# Autodesk Inventor assembly: Sestava
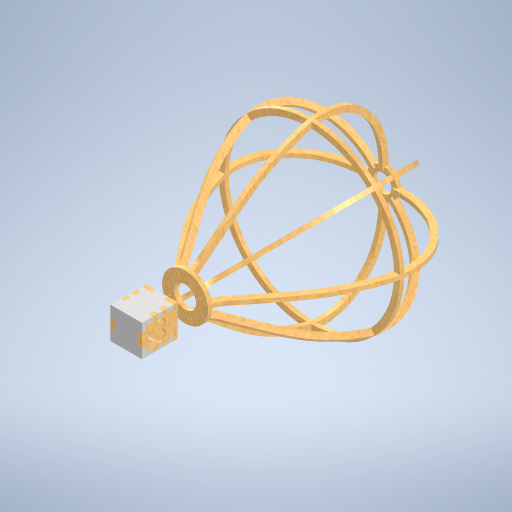
[picture p0: Inventor's stored thumbnail of the model, 512x512]
Saved by Autodesk Inventor 2023 (Build 270158000, 158)
## iProperties
Created: 2022-12-16
Part Number: Sestava
Document SubType Name: Assembly
Designer: David Zindović
Author: David Zindović
## Documents named in this file (9)
- C:\Users\David Zindović\Desktop\Projekti\Darila\Dekoracija - Balon za mami\Sestava.iam
- C:\Users\David Zindović\Desktop\Projekti\Darila\Dekoracija - Balon za mami\Sirsi obroc.ipt
- C:\Users\David Zindović\Desktop\Projekti\Darila\Dekoracija - Balon za mami\Balon skelet.ipt
- C:\Users\David Zindović\Desktop\Projekti\Darila\Dekoracija - Balon za mami\Vrhnji obrok.ipt
- C:\Users\David Zindović\Desktop\Projekti\Darila\Dekoracija - Balon za mami\Spodnji obroc.ipt
- C:\Users\David Zindović\Desktop\Projekti\Darila\Dekoracija - Balon za mami\Spodnji del - stranica.ipt
- C:\Users\David Zindović\Desktop\Projekti\Darila\Dekoracija - Balon za mami\Spodnji del - Drzalo za pismo.ipt
- C:\Users\David Zindović\Desktop\Projekti\Darila\Dekoracija - Balon za mami\Stran Stran.ipt
- C:\Users\David Zindović\Desktop\Projekti\Darila\Dekoracija - Balon za mami\Spodi Spodnji.ipt
## Components (17 placed, 8 different names)
1. Sirsi obroc:1 — Mate:1, Mate:2, Mate:3, Mate:4, Mate:5, Mate:6, Mate:7, Mate:8, Mate:9, Mate:10, Mate:11, Mate:12, Mate:13, Mate:14, Mate:15, Mate:16, Mate:17, Mate:18, Mate:19, Mate:20, Mate:21, Mate:22, Mate:23, Mate:24
2. Balon skelet:1 — Mate:8, Mate:16, Mate:20, Mate:31
3. Balon skelet:2 — Mate:7, Mate:14, Mate:22
4. Balon skelet:3 — Mate:4, Mate:10, Mate:11
5. Balon skelet:4 — Mate:3, Mate:15, Mate:21
6. Balon skelet:5 — Mate:2, Mate:17, Mate:19, Mate:30
7. Balon skelet:6 — Mate:5, Mate:18, Mate:24, Mate:32
8. Balon skelet:7 — Mate:1, Mate:9, Mate:12
9. Balon skelet:8 — Mate:6, Mate:13, Mate:23, Mate:29, Flush:1
10. Vrhnji obrok:1 — Mate:29, Mate:30
11. Spodnji obroc:1 — Mate:31, Mate:32, Flush:1
12. Spodnji del - stranica:1 — Mate:35, Mate:36, Flush:3, Flush:8, Flush:9
13. Spodnji del - stranica:2 — Mate:33, Flush:2, Mate:34
14. Spodnji del - Drzalo za pismo:1 — Mate:33, Flush:2, Mate:34, Mate:35, Mate:36, Flush:3, Mate:37, Flush:4, Flush:5, Mate:38, Flush:6, Flush:7
15. Stran Stran:1 — Mate:37, Flush:4, Flush:5
16. Stran Stran:2 — Mate:38, Flush:6, Flush:7, Flush:10
17. Spodi Spodnji:1 — Flush:8, Flush:9, Flush:10
## Relationships (44: Mate 34, Flush 10)
- Mate:1: Sirsi obroc:1 ↔ Balon skelet:7
- Mate:2: Sirsi obroc:1 ↔ Balon skelet:5
- Mate:3: Sirsi obroc:1 ↔ Balon skelet:4
- Mate:4: Sirsi obroc:1 ↔ Balon skelet:3
- Mate:5: Sirsi obroc:1 ↔ Balon skelet:6
- Mate:6: Sirsi obroc:1 ↔ Balon skelet:8
- Mate:7: Sirsi obroc:1 ↔ Balon skelet:2
- Mate:8: Sirsi obroc:1 ↔ Balon skelet:1
- Mate:9: Sirsi obroc:1 ↔ Balon skelet:7
- Mate:10: Sirsi obroc:1 ↔ Balon skelet:3
- Mate:11: Sirsi obroc:1 ↔ Balon skelet:3
- Mate:12: Sirsi obroc:1 ↔ Balon skelet:7
- Mate:13: Sirsi obroc:1 ↔ Balon skelet:8
- Mate:14: Sirsi obroc:1 ↔ Balon skelet:2
- Mate:15: Sirsi obroc:1 ↔ Balon skelet:4
- Mate:16: Sirsi obroc:1 ↔ Balon skelet:1
- Mate:17: Sirsi obroc:1 ↔ Balon skelet:5
- Mate:18: Sirsi obroc:1 ↔ Balon skelet:6
- Mate:19: Sirsi obroc:1 ↔ Balon skelet:5
- Mate:20: Sirsi obroc:1 ↔ Balon skelet:1
- Mate:21: Sirsi obroc:1 ↔ Balon skelet:4
- Mate:22: Sirsi obroc:1 ↔ Balon skelet:2
- Mate:23: Sirsi obroc:1 ↔ Balon skelet:8
- Mate:24: Sirsi obroc:1 ↔ Balon skelet:6
- Mate:29: Balon skelet:8 ↔ Vrhnji obrok:1
- Mate:30: Balon skelet:5 ↔ Vrhnji obrok:1
- Mate:31: Balon skelet:1 ↔ Spodnji obroc:1
- Mate:32: Balon skelet:6 ↔ Spodnji obroc:1
- Flush:1: Balon skelet:8 ↔ Spodnji obroc:1
- Mate:33: Spodnji del - stranica:2 ↔ Spodnji del - Drzalo za pismo:1
- Flush:2: Spodnji del - stranica:2 ↔ Spodnji del - Drzalo za pismo:1
- Mate:34: Spodnji del - stranica:2 ↔ Spodnji del - Drzalo za pismo:1
- Mate:35: Spodnji del - stranica:1 ↔ Spodnji del - Drzalo za pismo:1
- Mate:36: Spodnji del - stranica:1 ↔ Spodnji del - Drzalo za pismo:1
- Flush:3: Spodnji del - stranica:1 ↔ Spodnji del - Drzalo za pismo:1
- Mate:37: Spodnji del - Drzalo za pismo:1 ↔ Stran Stran:1
- Flush:4: Spodnji del - Drzalo za pismo:1 ↔ Stran Stran:1
- Flush:5: Spodnji del - Drzalo za pismo:1 ↔ Stran Stran:1
- Mate:38: Spodnji del - Drzalo za pismo:1 ↔ Stran Stran:2
- Flush:6: Spodnji del - Drzalo za pismo:1 ↔ Stran Stran:2
- Flush:7: Spodnji del - Drzalo za pismo:1 ↔ Stran Stran:2
- Flush:8: Spodnji del - stranica:1 ↔ Spodi Spodnji:1
- Flush:9: Spodnji del - stranica:1 ↔ Spodi Spodnji:1
- Flush:10: Stran Stran:2 ↔ Spodi Spodnji:1
